# Autodesk Inventor assembly: podwojne koło zebate drugi skręt
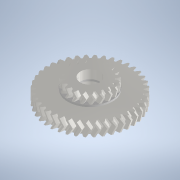
[picture p0: Inventor's stored thumbnail of the model, 180x180]
Saved by Autodesk Inventor 2021 (Build 250183000, 183)
## iProperties
Created: 2021-06-27
Part Number: podwojne koło zebate drugi skręt
Document SubType Name: Assembly
Designer: Łukasz
Author: Łukasz
## Documents named in this file (4)
- E:\GITHUB_Czołg\Szybki-Czolg-antyRadziecki\koła zębate\Design Accelerator\podwojne koło zebate drugi skręt.iam
- E:\GITHUB_Czołg\Szybki-Czolg-antyRadziecki\koła zębate\Design Accelerator\inny set zebow\Design Accelerator\Spur Gear11.ipt
- E:\GITHUB_Czołg\Szybki-Czolg-antyRadziecki\koła zębate\Design Accelerator\inny set zebow\Design Accelerator\Spur Gear21 bez spacera.ipt
- E:\GITHUB_Czołg\Szybki-Czolg-antyRadziecki\podkładka.ipt
## Components (3 placed, 3 different names)
1. Spur Gear1:1 — Rigid:1
2. Spur Gear2:1 — Rigid:2
3. podkładka:1 — Rigid:1, Rigid:2
## Relationships (2: WeldJoint 2)
- Rigid:1 [WeldJoint]: Spur Gear1:1 ↔ podkładka:1
- Rigid:2 [WeldJoint]: Spur Gear2:1 ↔ podkładka:1
